# Autodesk Inventor assembly: daVinci_Head_Assembly
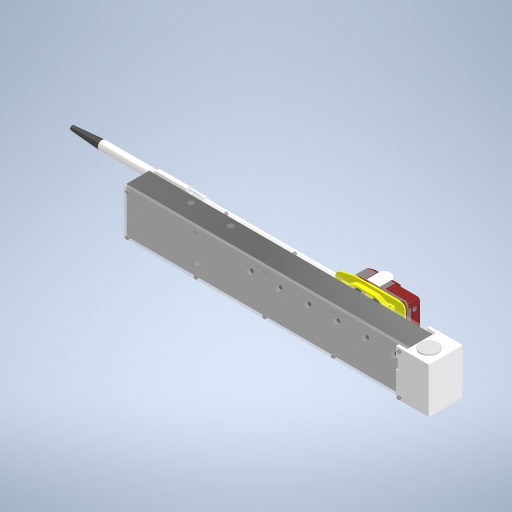
[picture p0: Inventor's stored thumbnail of the model, 512x512]
Saved by Autodesk Inventor 2024 (Build 280153000, 153)
## iProperties
Created: 2022-08-11
Part Number: daVinci_Head_Assembly
Document SubType Name: Assembly
Designer: alexw
Mass: 1326.84 g
Surface Area: 4941.83 cm^2
Volume: 1268.58 cm^3
Author: alexw
## Documents named in this file (4)
- C:\Users\AEWALDER\Documents\Inventor\03_CurrentProjects\MasterThesis\PSM_V1_Rillenkugellager\Ueberarbeiteter DaVincikopf\daVinci_Head_Assembly.iam
- C:\Users\AEWALDER\Documents\Inventor\03_CurrentProjects\MasterThesis\PSM_V1_Rillenkugellager\Ueberarbeiteter DaVincikopf\daVinciHead_FrameWork.iam
- C:\Users\AEWALDER\Documents\Inventor\03_CurrentProjects\MasterThesis\PSM_V1_Rillenkugellager\Ueberarbeiteter DaVincikopf\daVinciHead_Sled.iam
- C:\Users\AEWALDER\Documents\Inventor\03_CurrentProjects\MasterThesis\PSM_V1_Rillenkugellager\Riemen_Design_Assitant.ipt
## Components (3 placed, 3 different names)
1. daVinciHead_FrameWork:1 [sub-assembly] — Fluchtend:1, Fluchtend:2, Fluchtend:3, Passend:1, Tangential:1, Tangential:2, CarriageHub
2. daVinciHead_Sled:1 [sub-assembly] — Passend:1, Tangential:1, Tangential:2, CarriageHub
3. Riemen_Design_Assitant:1
## Relationships (7: Flush 3, Mate 2, Tangent 2)
- Fluchtend:1 [Flush]: daVinciHead_FrameWork:1
- Fluchtend:2 [Flush]: daVinciHead_FrameWork:1
- Fluchtend:3 [Flush]: daVinciHead_FrameWork:1
- Passend:1 [Mate]: daVinciHead_FrameWork:1 ↔ daVinciHead_Sled:1
- Tangential:1: daVinciHead_FrameWork:1 ↔ daVinciHead_Sled:1
- Tangential:2: daVinciHead_FrameWork:1 ↔ daVinciHead_Sled:1
- CarriageHub [Mate] (20 mm): daVinciHead_FrameWork:1 ↔ daVinciHead_Sled:1
